# Autodesk Inventor assembly: 3136 1133 84
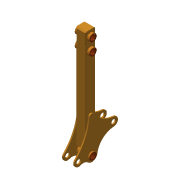
[picture p0: Inventor's stored thumbnail of the model, 180x180]
Saved by Autodesk Inventor 2022 Beta2 (Build 260130000, 130) ContinuousBuild 0
## iProperties
Shininess: 64.0
Length Units: 11269
Angle Units: 11279
Time Units: 11290
Mass Units: 11283
Length Display Precision: 3
Angle Display Precision: 2
Compacted: True
Created: 2003-04-13
Part Number: 3136 1133 84
Document SubType Name: Assembly
Designer: Uffe Bak
Density: 0.0
Volumn: 0.0
Area: 0.0
PropertySet Name: Model Information
Control State: 0
Master: False
Checked Out: False
Author: Uffe Bak
## Documents named in this file (7)
- C:\Autodesk Inventor 2021 Intro Practice Files\BOM\3136 1133 84.iam
- C:\Autodesk Inventor 2021 Intro Practice Files\BOM\3136 1094 55.ipt
- C:\Autodesk Inventor 2021 Intro Practice Files\BOM\3136 1133 85.ipt
- C:\Autodesk Inventor 2021 Intro Practice Files\BOM\3136 1094 56.ipt
- C:\Autodesk Inventor 2021 Intro Practice Files\BOM\3136 1094 58.ipt
- C:\Autodesk Inventor 2021 Intro Practice Files\BOM\3136 1144 21.ipt
- C:\Autodesk Inventor 2021 Intro Practice Files\BOM\0500 4500 24.ipt
## Components (14 placed, 6 different names)
1. 3136 1094 55:1 — Flush:1, Mate:1, Mate:2, Mate:3, Mate:4, Flush:2, Flush:3, Flush:4, Flush:5, Mate:7, Mate:8, Insert:1
2. 3136 1133 85:1 — Flush:1, Mate:1, Mate:2, Mate:3, Mate:5, Mate:6
3. 3136 1133 85:2 — Mate:4, Mate:5, Mate:6, Insert:3
4. 3136 1094 56:1 — Flush:2, Flush:3, Flush:4, Insert:2
5. 3136 1094 58:1 — Flush:5, Mate:7, Mate:8
6. 3136 1144 21:1 — Insert:1, Insert:5, Insert:9
7. 3136 1144 21:2 — Insert:3, Insert:4, Insert:7
8. 3136 1144 21:3 — Insert:2, Insert:6, Insert:8
9. 0500 4500 24:1 — Insert:4
10. 0500 4500 24:2 — Insert:8
11. 0500 4500 24:3 — Insert:5
12. 0500 4500 24:4 — Insert:9
13. 0500 4500 24:5 — Insert:6
14. 0500 4500 24:6 — Insert:7
## Relationships (22: Insert 9, Mate 8, Flush 5)
- Flush:1: 3136 1094 55:1 ↔ 3136 1133 85:1
- Mate:1 (50 mm): 3136 1094 55:1 ↔ 3136 1133 85:1
- Mate:2: 3136 1094 55:1 ↔ 3136 1133 85:1
- Mate:3: 3136 1094 55:1 ↔ 3136 1133 85:1
- Mate:4: 3136 1094 55:1 ↔ 3136 1133 85:2
- Mate:5: 3136 1133 85:1 ↔ 3136 1133 85:2
- Mate:6: 3136 1133 85:1 ↔ 3136 1133 85:2
- Flush:2: 3136 1094 55:1 ↔ 3136 1094 56:1
- Flush:3: 3136 1094 55:1 ↔ 3136 1094 56:1
- Flush:4: 3136 1094 55:1 ↔ 3136 1094 56:1
- Flush:5: 3136 1094 55:1 ↔ 3136 1094 58:1
- Mate:7: 3136 1094 55:1 ↔ 3136 1094 58:1
- Mate:8: 3136 1094 55:1 ↔ 3136 1094 58:1
- Insert:1 (-18.5 mm): 3136 1094 55:1 ↔ 3136 1144 21:1
- Insert:2 (18.5 mm): 3136 1094 56:1 ↔ 3136 1144 21:3
- Insert:3 (8.5 mm): 3136 1133 85:2 ↔ 3136 1144 21:2
- Insert:4: 3136 1144 21:2 ↔ 0500 4500 24:1
- Insert:5: 3136 1144 21:1 ↔ 0500 4500 24:3
- Insert:6: 3136 1144 21:3 ↔ 0500 4500 24:5
- Insert:7: 3136 1144 21:2 ↔ 0500 4500 24:6
- Insert:8: 3136 1144 21:3 ↔ 0500 4500 24:2
- Insert:9: 3136 1144 21:1 ↔ 0500 4500 24:4
